# Autodesk Inventor assembly: 射出_エンコーダーパーツ1
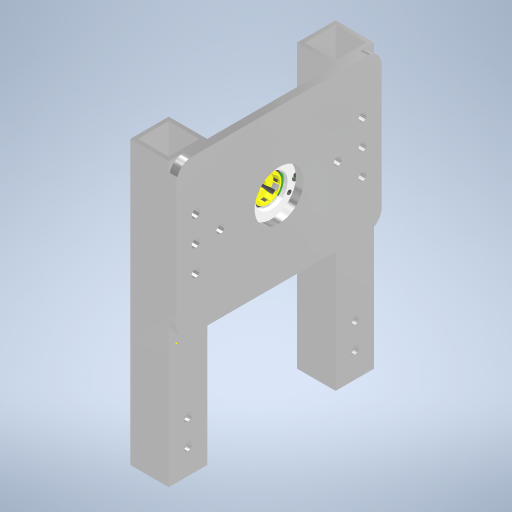
[picture p0: Inventor's stored thumbnail of the model, 512x512]
Saved by Autodesk Inventor 2023 (Build 270158000, 158)
## iProperties
Created: 2022-04-23
Part Number: 射出_エンコーダーパーツ1
Document SubType Name: Assembly
Designer: yuta
Author: yuta
## Documents named in this file (4)
- C:\Users\yuta\Documents\NHK\射出_エンコーダーパーツ1.iam
- C:\Users\yuta\Documents\NHK\射出_角柱6.ipt
- C:\Users\yuta\Documents\NHK\射出_エンコーダー固定2.ipt
- C:\Users\yuta\Documents\NHK\type1\amt102-v.iam
## Components (4 placed, 3 different names)
1. 射出_角柱6:1 — メイト:5, メイト:6, メイト:7
2. 射出_角柱6:2 — メイト:1, メイト:2, メイト:3, メイト:4
3. 射出_エンコーダー固定2:1 — メイト:1, メイト:2, メイト:3, メイト:4, メイト:5, メイト:6, メイト:7, メイト:8, メイト:9
4. amt102-v:2 [sub-assembly] — メイト:8, メイト:9
## Relationships (9: Mate 9)
- メイト:1 [Mate]: 射出_角柱6:2 ↔ 射出_エンコーダー固定2:1
- メイト:2 [Mate]: 射出_角柱6:2 ↔ 射出_エンコーダー固定2:1
- メイト:3 [Mate]: 射出_角柱6:2 ↔ 射出_エンコーダー固定2:1
- メイト:4 [Mate]: 射出_角柱6:2 ↔ 射出_エンコーダー固定2:1
- メイト:5 [Mate]: 射出_角柱6:1 ↔ 射出_エンコーダー固定2:1
- メイト:6 [Mate]: 射出_角柱6:1 ↔ 射出_エンコーダー固定2:1
- メイト:7 [Mate]: 射出_角柱6:1 ↔ 射出_エンコーダー固定2:1
- メイト:8 [Mate]: 射出_エンコーダー固定2:1 ↔ amt102-v:2
- メイト:9 [Mate]: 射出_エンコーダー固定2:1 ↔ amt102-v:2
